# Autodesk Inventor assembly: Kicker_assembly
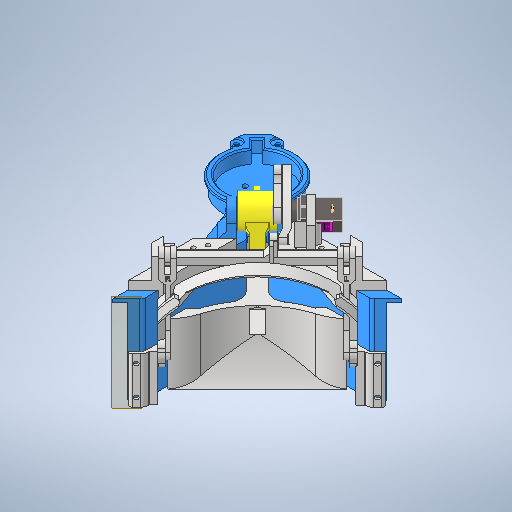
[picture p0: Inventor's stored thumbnail of the model, 512x512]
Saved by Autodesk Inventor 2025.1 (Build 291241000, 241)
## iProperties
Created: 2026-04-18
Part Number: Kicker_assembly
Document SubType Name: Assembly
Designer: User
Author: User
## Documents named in this file (14)
- D:\One Drive\OneDrive - Politeknik Sultan Salahuddin Abdul Aziz Shah\Documents\Inventor\RobosotPSA\Kicker_assembly.iam
- D:\One Drive\OneDrive - Politeknik Sultan Salahuddin Abdul Aziz Shah\Documents\Inventor\RobosotPSA\Kicker_v2.ipt
- D:\One Drive\OneDrive - Politeknik Sultan Salahuddin Abdul Aziz Shah\Documents\Inventor\RobosotPSA\Solenoid JF-0826B\Solenoid JF-0826B\Solenoid JF-0826B.ipt
- D:\One Drive\OneDrive - Politeknik Sultan Salahuddin Abdul Aziz Shah\Documents\Inventor\RobosotPSA\KickerRoll.ipt
- D:\One Drive\OneDrive - Politeknik Sultan Salahuddin Abdul Aziz Shah\Documents\Inventor\RobosotPSA\KickerFoot.ipt
- D:\One Drive\OneDrive - Politeknik Sultan Salahuddin Abdul Aziz Shah\Documents\Inventor\RobosotPSA\TheBall70mm.ipt
- D:\One Drive\OneDrive - Politeknik Sultan Salahuddin Abdul Aziz Shah\Documents\Inventor\RobosotPSA\DC Motor Speed Controller\DC Motor Speed Controller\DC Motor Speed Controller.ipt
- D:\One Drive\OneDrive - Politeknik Sultan Salahuddin Abdul Aziz Shah\Documents\Inventor\RobosotPSA\Dribbler_v1.ipt
- D:\One Drive\OneDrive - Politeknik Sultan Salahuddin Abdul Aziz Shah\Documents\Inventor\RobosotPSA\Assembly3.iam
- Dribbler_Type1.iam
- D:\One Drive\OneDrive - Politeknik Sultan Salahuddin Abdul Aziz Shah\Documents\Inventor\RobosotPSA\Dribbler_Type2.iam
- D:\One Drive\OneDrive - Politeknik Sultan Salahuddin Abdul Aziz Shah\Documents\Inventor\RobosotPSA\GripperAssy.iam
- D:\One Drive\OneDrive - Politeknik Sultan Salahuddin Abdul Aziz Shah\Documents\Inventor\RobosotPSA\KimiFrontCover.iam
- D:\One Drive\OneDrive - Politeknik Sultan Salahuddin Abdul Aziz Shah\Documents\Inventor\RobosotPSA\Dribbler_Type3.iam
## Components (12 placed, 12 different names)
1. Kicker_v2:1 — Mate:1, Mate:2, Mate:3, Flush:2, Mate:6, Mate:7, Mate:8, Mate:9, Mate:10
2. Solenoid JF-0826B:1 — Mate:1, Mate:2
3. KickerRoll:1 — Mate:3, Flush:1
4. KickerFoot:1 — Flush:1
5. TheBall70mm:1
6. DC Motor Speed Controller:1
7. Dribbler_v1:1 — Flush:2, Mate:4, Mate:5, Flush:3
8. Dribbler_Type1:1 [sub-assembly] — Mate:4, Mate:5
9. Dribbler_Type2:1 [sub-assembly] — Flush:3
10. GripperAssy:1 [sub-assembly] — Mate:6, Mate:7
11. KimiFrontCover:1 [sub-assembly]
12. Dribbler_Type3:1 [sub-assembly] — Mate:8, Mate:9, Mate:10
## Relationships (13: Mate 10, Flush 3)
- Mate:1: Kicker_v2:1 ↔ Solenoid JF-0826B:1
- Mate:2: Kicker_v2:1 ↔ Solenoid JF-0826B:1
- Mate:3: Kicker_v2:1 ↔ KickerRoll:1
- Flush:1: KickerRoll:1 ↔ KickerFoot:1
- Flush:2: Kicker_v2:1 ↔ Dribbler_v1:1
- Mate:4 (0.5 mm): Dribbler_v1:1 ↔ Dribbler_Type1:1
- Mate:5: Dribbler_v1:1 ↔ Dribbler_Type1:1
- Mate:6: Kicker_v2:1 ↔ GripperAssy:1
- Mate:7: Kicker_v2:1 ↔ GripperAssy:1
- Flush:3: Dribbler_v1:1 ↔ Dribbler_Type2:1
- Mate:8: Kicker_v2:1 ↔ Dribbler_Type3:1
- Mate:9: Kicker_v2:1 ↔ Dribbler_Type3:1
- Mate:10: Kicker_v2:1 ↔ Dribbler_Type3:1
